# Autodesk Inventor assembly: Jetson nano_fixed
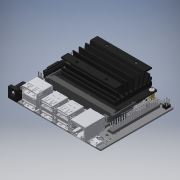
[picture p0: Inventor's stored thumbnail of the model, 180x180]
Saved by Autodesk Inventor 2019 (Build 230136000, 136)
## iProperties
Created: 2019-07-11
Part Number: Jetson nano_fixed
Material: Типовые
Document SubType Name: Assembly
Designer: Петров Иван
Sending System: Autodesk Translation Framework v8.2.0.1029
Preprocessor: ST-DEVELOPER v18
Title: C:/Users/Toby/Desktop/Jetson nano_fixed.step
## Documents named in this file (6)
- E:\IVAN\Ivan_desktop\My_projects\MyDrone\design\standart components\JetsonNano\Jetson nano_fixed.iam
- E:\IVAN\Ivan_desktop\My_projects\MyDrone\design\standart components\JetsonNano\142-13449-1000-A02_ASM.iam
- E:\IVAN\Ivan_desktop\My_projects\MyDrone\design\standart components\JetsonNano\PORG_HEX_STANDOFF.ipt
- E:\IVAN\Ivan_desktop\My_projects\MyDrone\design\standart components\JetsonNano\PORG_SYSTEM_SCREW.ipt
- E:\IVAN\Ivan_desktop\My_projects\MyDrone\design\standart components\JetsonNano\244-63448-0000-000_ASM.iam
- E:\IVAN\Ivan_desktop\My_projects\MyDrone\design\standart components\JetsonNano\155-0576-000.ipt
## Components (9 placed, 5 different names)
1. 142-13449-1000-A02_ASM:1 [sub-assembly] — Mate:1, Angle:1, Mate:2, Angle:2
2. PORG_HEX_STANDOFF:1
3. PORG_HEX_STANDOFF:2
4. PORG_SYSTEM_SCREW:1
5. PORG_SYSTEM_SCREW:2
6. 244-63448-0000-000_ASM:1 [sub-assembly]
7. PORG_SYSTEM_SCREW:3
8. PORG_SYSTEM_SCREW:4
9. 155-0576-000:1
## Relationships (4: Mate 2, Angle 2)
- Mate:1: 142-13449-1000-A02_ASM:1
- Angle:1 (0 deg): 142-13449-1000-A02_ASM:1
- Mate:2: 142-13449-1000-A02_ASM:1
- Angle:2 (0 deg): 142-13449-1000-A02_ASM:1
